# Autodesk Inventor assembly: anode-on-flange
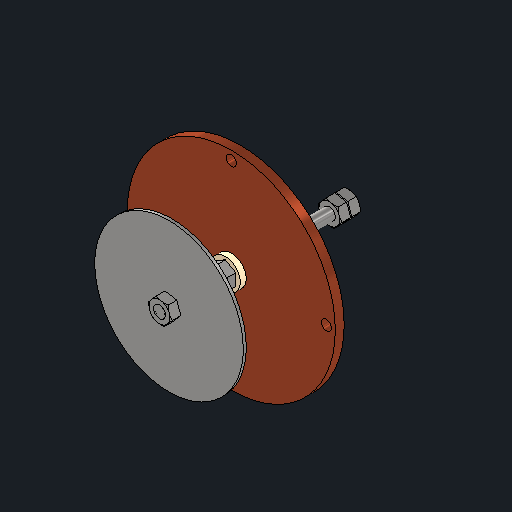
[picture p0: Inventor's stored thumbnail of the model, 512x512]
Saved by Autodesk Inventor 2026 (Build 300175050, 175E)
## iProperties
Created: 2024-05-20
Part Number: anode-on-flange
Document SubType Name: Assembly
Designer: queezz
Author: queezz
## Documents named in this file (7)
- C:\Users\queez\Dropbox\Drawings\PIHTI\Plasma Vessel\Plasma-Box\anode-on-flange.iam
- C:\Users\queez\Dropbox\Drawings\PIHTI\Plasma Vessel\Plasma-Box\anode_holder.ipt
- C:\Users\queez\Dropbox\Drawings\PIHTI\Plasma Vessel\Plasma-Box\anode-disk.ipt
- C:\Users\queez\Dropbox\Drawings\PIHTI\Plasma Vessel\Plasma-Box\anode-m4-threaded-rod.ipt
- C:\Users\queez\Dropbox\Drawings\PIHTI\ContentCenter\Ceramics\ceramic_washer_M4.ipt
- C:\Users\queez\Dropbox\Drawings\PIHTI\ContentCenter\Ceramics\ceramic_bushing_M4.ipt
- C:\Users\queez\Dropbox\Drawings\PIHTI\ContentCenter\Fastners\M4-nut.ipt
## Components (11 placed, 6 different names)
1. anode_holder:1 — Mate:1, Flush:1, Mate:2, Rigid:1, Rigid:2, Mate:3, Mate:4, Mate:5
2. anode-disk:1 — Mate:4, Rigid:6, Rigid:3, Mate:5
3. anode-m4-threaded-rod:1 — Mate:3, Rigid:9, Rigid:7
4. ceramic_washer_M4:1 — Rigid:2, Rigid:4
5. ceramic_bushing_M4:1 — Rigid:1, Rigid:5
6. JIS B 1181 -finished Class 1 - Metric Class 1 -finishedM4:1 — Rigid:6, Rigid:7
7. JIS B 1181 -finished Class 1 - Metric Class 1 -finishedM4:2 — Rigid:3
8. JIS B 1181 -finished Class 1 - Metric Class 1 -finishedM4:3 — Rigid:4
9. JIS B 1181 -finished Class 1 - Metric Class 1 -finishedM4:4 — Rigid:5
10. JIS B 1181 -finished Class 1 - Metric Class 1 -finishedM4:5 — Rigid:8
11. JIS B 1181 -finished Class 1 - Metric Class 1 -finishedM4:6 — Rigid:9, Rigid:8
## Relationships (15: WeldJoint 9, Mate 5, Flush 1)
- Mate:1: anode_holder:1
- Flush:1: anode_holder:1
- Mate:2: anode_holder:1
- Rigid:1 [WeldJoint]: anode_holder:1 ↔ ceramic_bushing_M4:1
- Rigid:2 [WeldJoint]: anode_holder:1 ↔ ceramic_washer_M4:1
- Mate:3: anode_holder:1 ↔ anode-m4-threaded-rod:1
- Mate:4: anode_holder:1 ↔ anode-disk:1
- Rigid:6 [WeldJoint]: anode-disk:1 ↔ JIS B 1181 -finished Class 1 - Metric Class 1 -finishedM4:1
- Rigid:3 [WeldJoint]: anode-disk:1 ↔ JIS B 1181 -finished Class 1 - Metric Class 1 -finishedM4:2
- Rigid:4 [WeldJoint]: ceramic_washer_M4:1 ↔ JIS B 1181 -finished Class 1 - Metric Class 1 -finishedM4:3
- Rigid:5 [WeldJoint]: ceramic_bushing_M4:1 ↔ JIS B 1181 -finished Class 1 - Metric Class 1 -finishedM4:4
- Rigid:9 [WeldJoint] (-1 mm): anode-m4-threaded-rod:1 ↔ JIS B 1181 -finished Class 1 - Metric Class 1 -finishedM4:6
- Rigid:8 [WeldJoint] (0.4 mm): JIS B 1181 -finished Class 1 - Metric Class 1 -finishedM4:5 ↔ JIS B 1181 -finished Class 1 - Metric Class 1 -finishedM4:6
- Rigid:7 [WeldJoint]: anode-m4-threaded-rod:1 ↔ JIS B 1181 -finished Class 1 - Metric Class 1 -finishedM4:1
- Mate:5 (20 mm): anode_holder:1 ↔ anode-disk:1
